# Autodesk Inventor assembly: Assembly_Opentrons_opticsmodule
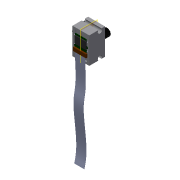
[picture p0: Inventor's stored thumbnail of the model, 180x180]
Saved by Autodesk Inventor 2019.4 (Build 234330000, 330)
## iProperties
Created: 2020-10-20
Part Number: Assembly_Opentrons_opticsmodule
Document SubType Name: Assembly
Designer: diederichbenedict
Author: diederichbenedict
## Documents named in this file (5)
- C:\Users\diederichbenedict\Dropbox\Dokumente\Promotion\PROJECTS\OPENTRONS\INVENTOR\Assembly_Opentrons_opticsmodule.iam
- C:\Users\diederichbenedict\Dropbox\Dokumente\Promotion\PROJECTS\OPENTRONS\INVENTOR\00_Z_Focus_CCTV_Camera.ipt
- C:\Users\diederichbenedict\Dropbox\Dokumente\Promotion\PROJECTS\OPENTRONS\INVENTOR\00_CCTV_Fisheye_Starlight_f2.8mm_Fno_1.4.ipt
- C:\Users\diederichbenedict\Dropbox\Dokumente\Promotion\PROJECTS\OPENTRONS\INVENTOR\00_RasPi_Camera.ipt
- C:\Users\diederichbenedict\Dropbox\Dokumente\Promotion\PROJECTS\OPENTRONS\INVENTOR\01_Adapter_Raspicam_CCTV_lens.ipt
## Components (4 placed, 4 different names)
1. 00_Z_Focus_CCTV_Camera:1
2. 00_CCTV_Fisheye_Starlight_f2.8mm_Fno_1.4:1
3. 01_Adapter_Raspicam_CCTV_lens:1
4. 00_RasPi_Camera:1
## Relationships (7: Mate 4, Flush 2, Angle 1)
- [Mate]: 00_Z_Focus_CCTV_Camera:1 ↔ 00_CCTV_Fisheye_Starlight_f2.8mm_Fno_1.4:1
- [Mate] (-33 mm): 00_Z_Focus_CCTV_Camera:1 ↔ 00_CCTV_Fisheye_Starlight_f2.8mm_Fno_1.4:1
- [Mate]: 00_CCTV_Fisheye_Starlight_f2.8mm_Fno_1.4:1 ↔ 00_RasPi_Camera:1
- [Angle] (0 deg): 00_Z_Focus_CCTV_Camera:1 ↔ 00_RasPi_Camera:1
- [Mate] (2 mm): 00_Z_Focus_CCTV_Camera:1 ↔ 00_RasPi_Camera:1
- [Flush]: 00_Z_Focus_CCTV_Camera:1 ↔ 01_Adapter_Raspicam_CCTV_lens:1
- [Flush]: 00_Z_Focus_CCTV_Camera:1 ↔ 01_Adapter_Raspicam_CCTV_lens:1
